# Autodesk Inventor assembly: PCB chip
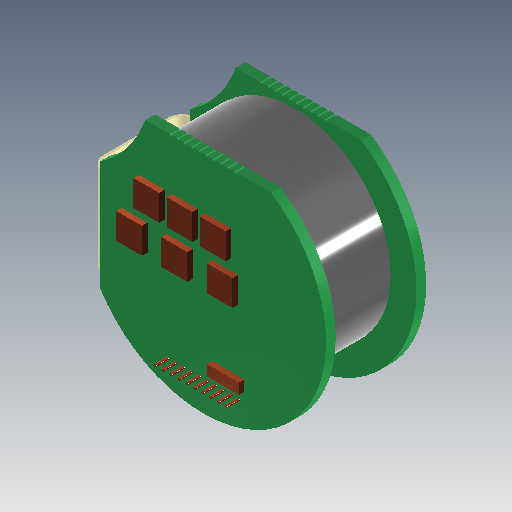
[picture p0: Inventor's stored thumbnail of the model, 512x512]
Saved by Autodesk Inventor 2020.3 (Build 243373010, 373A)
## iProperties
Created: 2021-04-10
Part Number: PCB chip
Document SubType Name: Assembly
Designer: marti
Mass: 10.6825 g
Surface Area: 79.7111 cm^2
Volume: 11.6908 cm^3
Density: 0.913754 g/cm^3
Author: marti
## Documents named in this file (5)
- C:\Users\marti\Documents\Inventor\RobotManipulateArm\17.4.2021 - Complete new IDEA\Servo\PCB chip.iam
- C:\Users\marti\Documents\Inventor\RobotManipulateArm\17.4.2021 - Complete new IDEA\Servo\PCB od servo motor.ipt
- C:\Users\marti\Documents\Inventor\RobotManipulateArm\17.4.2021 - Complete new IDEA\Servo\PCB of servo motor 2.ipt
- C:\Users\marti\Documents\Inventor\RobotManipulateArm\17.4.2021 - Complete new IDEA\Servo\Thermal pad.ipt
- C:\Users\marti\Documents\Inventor\RobotManipulateArm\New parts\Connecting cable.ipt
## Components (4 placed, 4 different names)
1. PCB od servo motor:2 — Flush:1, Mate:1, Mate:2, Mate:3, Mate:4, Flush:2, Mate:5, Mate:7, Mate:10, Mate:11, Mate:12
2. PCB of servo motor 2:1 — Mate:4, Flush:2, Mate:5, Mate:6, Mate:8
3. Thermal pad:1 — Mate:6, Mate:7, Mate:8
4. Connecting cable:1 — Mate:10, Mate:11, Mate:12
## Relationships (13: Mate 11, Flush 2)
- Flush:1: PCB od servo motor:2
- Mate:1: PCB od servo motor:2
- Mate:2: PCB od servo motor:2
- Mate:3: PCB od servo motor:2
- Mate:4 (12.5 mm): PCB od servo motor:2 ↔ PCB of servo motor 2:1
- Flush:2: PCB od servo motor:2 ↔ PCB of servo motor 2:1
- Mate:5: PCB od servo motor:2 ↔ PCB of servo motor 2:1
- Mate:6: PCB of servo motor 2:1 ↔ Thermal pad:1
- Mate:7: PCB od servo motor:2 ↔ Thermal pad:1
- Mate:8: PCB of servo motor 2:1 ↔ Thermal pad:1
- Mate:10: PCB od servo motor:2 ↔ Connecting cable:1
- Mate:11: PCB od servo motor:2 ↔ Connecting cable:1
- Mate:12: PCB od servo motor:2 ↔ Connecting cable:1
